# Autodesk Inventor assembly: monitor blanking
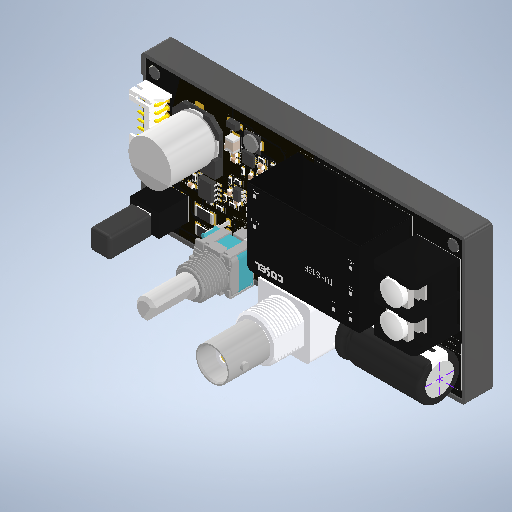
[picture p0: Inventor's stored thumbnail of the model, 512x512]
Saved by Autodesk Inventor 2025.3 (Build 293356000, 356)
## iProperties
Created: 2025-05-23
Part Number: monitor blanking
Document SubType Name: Assembly
Designer: Yuhsuan Chen
Author: Yuhsuan Chen
## Documents named in this file (5)
- C:\Users\Yuhsuan Chen\Desktop\ME\Monitor blanking\Source\monitor blanking Master.iam
- C:\Users\Yuhsuan Chen\Desktop\ME\Monitor blanking\Source\PCBA\Monitor_Blanking_V3.iam
- C:\Users\Yuhsuan Chen\Desktop\ME\Monitor blanking\Source\base.ipt
- C:\Users\Yuhsuan Chen\Desktop\ME\Monitor blanking\Source\Button.ipt
- C:\Users\Public\Documents\Autodesk\Inventor 2025\Part3.ipt
## Components (4 placed, 4 different names)
1. Monitor_Blanking_V3:1 [sub-assembly] — Insert:1, Mate:1, Mate:2, Flush:1
2. base:1 — Insert:1
3. Button:1 — Mate:1, Mate:2
4. Part3:1 — Flush:1
## Relationships (4: Mate 2, Insert 1, Flush 1)
- Insert:1 (-0.2 mm): Monitor_Blanking_V3:1 ↔ base:1
- Mate:1 (1 mm): Monitor_Blanking_V3:1 ↔ Button:1
- Mate:2: Monitor_Blanking_V3:1 ↔ Button:1
- Flush:1: Monitor_Blanking_V3:1 ↔ Part3:1
